# Autodesk Inventor assembly: Quick Assembly
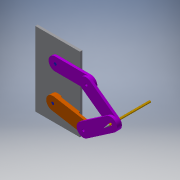
[picture p0: Inventor's stored thumbnail of the model, 180x180]
Saved by Autodesk Inventor 2017 (Build 210142000, 142)
## iProperties
Created: 2017-04-26
Part Number: Quick Assembly
Document SubType Name: Assembly
Designer: Parshant Bombhi
Author: Parshant Bombhi
## Documents named in this file (8)
- C:\Users\Parshant Bombhi\sfuvault\Rembrant Robotics\Parshant Files\Quick Assembly.iam
- C:\Users\Parshant Bombhi\sfuvault\Rembrant Robotics\Parshant Files\8.5 x 11 paper.ipt
- C:\Users\Parshant Bombhi\sfuvault\Rembrant Robotics\Parshant Files\Base.ipt
- C:\Users\Parshant Bombhi\sfuvault\Rembrant Robotics\Parshant Files\Inner Arm Thin.ipt
- C:\Users\Parshant Bombhi\sfuvault\Rembrant Robotics\Parshant Files\Inner Arm Thick.ipt
- C:\Users\Parshant Bombhi\sfuvault\Rembrant Robotics\Parshant Files\Pencil\pencil_assembly.iam
- C:\Users\Parshant Bombhi\sfuvault\Rembrant Robotics\Parshant Files\608.ipt
- C:\Users\Parshant Bombhi\sfuvault\Rembrant Robotics\Parshant Files\8mm Shaft.ipt
## Components (11 placed, 7 different names)
1. 8.5 x 11 paper:1 — Mate:1, Flush:1, Flush:2
2. Base:1 — Mate:1, Flush:1, Flush:2, Mate:2, Mate:3, Mate:8, Mate:9, Mate:13, Flush:15, Mate:16, Flush:16
3. Inner Arm Thin:1 — Mate:6, Mate:7, Mate:8, Mate:9, Flush:18
4. Inner Arm Thin:2 — Mate:6, Mate:7, Mate:10, Mate:11, Flush:3
5. Inner Arm Thin:3 — Mate:4, Mate:10, Mate:20
6. Inner Arm Thick:1 — Mate:2, Mate:3, Mate:4, Flush:19, Mate:20
7. pencil_assembly:1 [sub-assembly] — Mate:11, Flush:3
8. 608:2 — Mate:13, Flush:15, Mate:19
9. 608:3 — Mate:16, Flush:16, Mate:18
10. 8mm Shaft:1 — Mate:18, Flush:18
11. 8mm Shaft:2 — Mate:19, Flush:19
## Relationships (22: Mate 15, Flush 7)
- Mate:1 (50 mm): 8.5 x 11 paper:1 ↔ Base:1
- Flush:1: 8.5 x 11 paper:1 ↔ Base:1
- Flush:2 (74 mm): 8.5 x 11 paper:1 ↔ Base:1
- Mate:2: Base:1 ↔ Inner Arm Thick:1
- Mate:3: Base:1 ↔ Inner Arm Thick:1
- Mate:4: Inner Arm Thin:3 ↔ Inner Arm Thick:1
- Mate:6: Inner Arm Thin:1 ↔ Inner Arm Thin:2
- Mate:7: Inner Arm Thin:1 ↔ Inner Arm Thin:2
- Mate:8: Base:1 ↔ Inner Arm Thin:1
- Mate:9: Base:1 ↔ Inner Arm Thin:1
- Mate:10: Inner Arm Thin:2 ↔ Inner Arm Thin:3
- Mate:11: Inner Arm Thin:2 ↔ pencil_assembly:1
- Flush:3 (-101 mm): Inner Arm Thin:2 ↔ pencil_assembly:1
- Mate:13: Base:1 ↔ 608:2
- Flush:15: Base:1 ↔ 608:2
- Mate:16: Base:1 ↔ 608:3
- Flush:16: Base:1 ↔ 608:3
- Mate:18: 608:3 ↔ 8mm Shaft:1
- Flush:18: Inner Arm Thin:1 ↔ 8mm Shaft:1
- Mate:19: 608:2 ↔ 8mm Shaft:2
- Flush:19: Inner Arm Thick:1 ↔ 8mm Shaft:2
- Mate:20: Inner Arm Thin:3 ↔ Inner Arm Thick:1
## Named parameters: DistanceFromPaperToBase = 50 mm, DistanceOfHolesFromEdge = 60 mm, LengthOfArm_Thicker = 135 mm, Thickness_Thicker = 14 mm, LengthOfArm_Thiner = 135 mm, Thickness_Thiner = 7 mm
